# Autodesk Inventor assembly: ElectricSkateboard
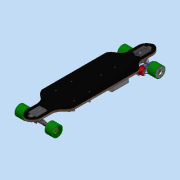
[picture p0: Inventor's stored thumbnail of the model, 180x180]
Saved by Autodesk Inventor 2015 SP1 (Build 190203100, 203)
## iProperties
Created: 2015-06-16
Part Number: ElectricSkateboard
Document SubType Name: Assembly
Designer: YOUR_NAME_HERE
Author: YOUR_NAME_HERE
## Documents named in this file (6)
- C:\Users\Rahul\Electric Skateboard\Electric Skateboard CAD\ElectricSkateboard.iam
- C:\Users\Rahul\Electric Skateboard\Electric Skateboard CAD\LongboardBare.iam
- C:\Users\Rahul\Electric Skateboard\Electric Skateboard CAD\MotorMountAssembly.iam
- C:\Users\Rahul\Electric Skateboard\Electric Skateboard CAD\Electronics_Assy.iam
- C:\Users\Rahul\Electric Skateboard\Electric Skateboard CAD\BatteryBox.ipt
- C:\Users\Rahul\Electric Skateboard\Electric Skateboard CAD\ArmingKeySlot.ipt
## Components (5 placed, 5 different names)
1. LongboardBare:1 [sub-assembly] — Mate:1, Mate:2, Flush:1, Flush:2, Flush:3, Angle:1, Tangent:1, Mate:3, Mate:4, Mate:6, Mate:7, Flush:6, Mate:8
2. MotorMountAssembly:1 [sub-assembly] — Mate:1, Mate:2
3. Electronics_Assy:1 [sub-assembly] — Flush:4, Mate:3, Mate:4
4. BatteryBox:1 — Flush:5, Mate:6, Mate:7
5. ArmingKeySlot:1 — Flush:6, Mate:8
## Relationships (15: Mate 7, Flush 6, Angle 1, Tangent 1)
- Mate:1: LongboardBare:1 ↔ MotorMountAssembly:1
- Mate:2: LongboardBare:1 ↔ MotorMountAssembly:1
- Flush:1: LongboardBare:1
- Flush:2: LongboardBare:1
- Flush:3: LongboardBare:1
- Angle:1 (0 deg): LongboardBare:1
- Tangent:1: LongboardBare:1
- Flush:4: Electronics_Assy:1
- Mate:3: LongboardBare:1 ↔ Electronics_Assy:1
- Mate:4: LongboardBare:1 ↔ Electronics_Assy:1
- Flush:5: BatteryBox:1
- Mate:6: LongboardBare:1 ↔ BatteryBox:1
- Mate:7: LongboardBare:1 ↔ BatteryBox:1
- Flush:6: LongboardBare:1 ↔ ArmingKeySlot:1
- Mate:8: LongboardBare:1 ↔ ArmingKeySlot:1
